# Autodesk Inventor assembly: robot_base
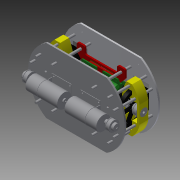
[picture p0: Inventor's stored thumbnail of the model, 180x180]
Saved by Autodesk Inventor 2014 SP1 (Build 180222100, 222)
## iProperties
Created: 2015-07-19
Part Number: robot_base
Document SubType Name: Assembly
Designer: astralien3000
Author: astralien3000
## Documents named in this file (8)
- C:\Users\astralien3000\Desktop\ceres\meca\v2016\robot_base.iam
- C:\Users\astralien3000\Desktop\ceres\meca\v2016\base.ipt
- C:\Users\astralien3000\Desktop\ceres\meca\v2016\odometer_block.iam
- C:\Users\astralien3000\Desktop\ceres\meca\v2016\wheel_block.iam
- C:\Users\astralien3000\Desktop\ceres\meca\lib\struct\vis_6mm_100mm.ipt
- C:\Users\astralien3000\Desktop\ceres\meca\lib\struct\patin_d18mm_e6mm.ipt
- C:\Users\astralien3000\Desktop\ceres\meca\v2016\motor.iam
- C:\Users\astralien3000\Desktop\ceres\meca\v2016\upper_base.ipt
## Components (23 placed, 7 different names)
1. base:1 — Placage:1, Affleurement:1, Placage:3, Placage:4, Placage:5, Placage:6, Placage:7, Placage:8, Placage:9, Placage:10, Placage:11, Placage:12, Placage:13, Placage:14, Placage:15, Placage:16, Placage:17, Placage:18, Placage:19, Placage:20, Placage:21, Placage:22, Placage:23, Placage:24, Placage:25, Placage:26, Placage:27, Placage:28, Placage:29, Placage:30, Placage:31, Placage:32, Placage:33, Placage:34, Placage:35, Placage:36, Placage:37, Placage:38, Placage:39, Placage:40, Placage:45
2. odometer_block:1 [sub-assembly] — Placage:3, Placage:4, Tangente:3
3. wheel_block:1 [sub-assembly] — Placage:5, Placage:6, Tangente:1
4. wheel_block:2 [sub-assembly] — Placage:7, Placage:8, Tangente:2
5. vis_6mm_100mm:1 — Placage:23, Placage:29
6. vis_6mm_100mm:2 — Placage:21, Placage:27
7. vis_6mm_100mm:3 — Placage:22, Placage:28
8. vis_6mm_100mm:4 — Placage:24, Placage:30
9. vis_6mm_100mm:5 — Placage:18, Placage:26
10. vis_6mm_100mm:6 — Placage:20, Placage:31, Placage:43
11. vis_6mm_100mm:7 — Placage:17, Placage:25, Placage:44
12. vis_6mm_100mm:8 — Placage:19, Placage:32
13. vis_6mm_100mm:9 — Placage:9, Placage:13
14. vis_6mm_100mm:10 — Placage:10, Placage:14
15. vis_6mm_100mm:11 — Placage:11, Placage:15
16. vis_6mm_100mm:12 — Placage:12, Placage:16
17. patin_d18mm_e6mm:1 — Placage:35, Placage:37
18. patin_d18mm_e6mm:2 — Placage:33, Placage:40, Tangente:2, Tangente:3
19. patin_d18mm_e6mm:3 — Placage:34, Placage:39, Tangente:1
20. patin_d18mm_e6mm:4 — Placage:36, Placage:38
21. motor:1 [sub-assembly] — Placage:49, Placage:50, Placage:51
22. motor:2 [sub-assembly] — Placage:46, Placage:47, Placage:48
23. upper_base:1 — Placage:43, Placage:44, Placage:45, Placage:46, Placage:47, Placage:48, Placage:49, Placage:50, Placage:51
## Relationships (52: Mate 48, Tangent 3, Flush 1)
- Placage:1 [Mate]: base:1
- Affleurement:1 [Flush]: base:1
- Placage:3 [Mate]: base:1 ↔ odometer_block:1
- Placage:4 [Mate]: base:1 ↔ odometer_block:1
- Placage:5 [Mate]: base:1 ↔ wheel_block:1
- Placage:6 [Mate]: base:1 ↔ wheel_block:1
- Placage:7 [Mate]: base:1 ↔ wheel_block:2
- Placage:8 [Mate]: base:1 ↔ wheel_block:2
- Placage:9 [Mate]: base:1 ↔ vis_6mm_100mm:9
- Placage:10 [Mate]: base:1 ↔ vis_6mm_100mm:10
- Placage:11 [Mate]: base:1 ↔ vis_6mm_100mm:11
- Placage:12 [Mate]: base:1 ↔ vis_6mm_100mm:12
- Placage:13 [Mate]: base:1 ↔ vis_6mm_100mm:9
- Placage:14 [Mate]: base:1 ↔ vis_6mm_100mm:10
- Placage:15 [Mate]: base:1 ↔ vis_6mm_100mm:11
- Placage:16 [Mate]: base:1 ↔ vis_6mm_100mm:12
- Placage:17 [Mate]: base:1 ↔ vis_6mm_100mm:7
- Placage:18 [Mate]: base:1 ↔ vis_6mm_100mm:5
- Placage:19 [Mate]: base:1 ↔ vis_6mm_100mm:8
- Placage:20 [Mate]: base:1 ↔ vis_6mm_100mm:6
- Placage:21 [Mate]: base:1 ↔ vis_6mm_100mm:2
- Placage:22 [Mate]: base:1 ↔ vis_6mm_100mm:3
- Placage:23 [Mate]: base:1 ↔ vis_6mm_100mm:1
- Placage:24 [Mate]: base:1 ↔ vis_6mm_100mm:4
- Placage:25 [Mate]: base:1 ↔ vis_6mm_100mm:7
- Placage:26 [Mate]: base:1 ↔ vis_6mm_100mm:5
- Placage:27 [Mate]: base:1 ↔ vis_6mm_100mm:2
- Placage:28 [Mate]: base:1 ↔ vis_6mm_100mm:3
- Placage:29 [Mate]: base:1 ↔ vis_6mm_100mm:1
- Placage:30 [Mate]: base:1 ↔ vis_6mm_100mm:4
- Placage:31 [Mate]: base:1 ↔ vis_6mm_100mm:6
- Placage:32 [Mate]: base:1 ↔ vis_6mm_100mm:8
- Placage:33 [Mate]: base:1 ↔ patin_d18mm_e6mm:2
- Placage:34 [Mate]: base:1 ↔ patin_d18mm_e6mm:3
- Placage:35 [Mate]: base:1 ↔ patin_d18mm_e6mm:1
- Placage:36 [Mate]: base:1 ↔ patin_d18mm_e6mm:4
- Placage:37 [Mate]: base:1 ↔ patin_d18mm_e6mm:1
- Placage:38 [Mate]: base:1 ↔ patin_d18mm_e6mm:4
- Placage:39 [Mate]: base:1 ↔ patin_d18mm_e6mm:3
- Placage:40 [Mate]: base:1 ↔ patin_d18mm_e6mm:2
- Tangente:1: wheel_block:1 ↔ patin_d18mm_e6mm:3
- Tangente:2: wheel_block:2 ↔ patin_d18mm_e6mm:2
- Tangente:3: odometer_block:1 ↔ patin_d18mm_e6mm:2
- Placage:43 [Mate]: vis_6mm_100mm:6 ↔ upper_base:1
- Placage:44 [Mate]: vis_6mm_100mm:7 ↔ upper_base:1
- Placage:45 [Mate] (80 mm): base:1 ↔ upper_base:1
- Placage:46 [Mate]: motor:2 ↔ upper_base:1
- Placage:47 [Mate]: motor:2 ↔ upper_base:1
- Placage:48 [Mate]: motor:2 ↔ upper_base:1
- Placage:49 [Mate]: motor:1 ↔ upper_base:1
- Placage:50 [Mate]: motor:1 ↔ upper_base:1
- Placage:51 [Mate]: motor:1 ↔ upper_base:1
